# Autodesk Inventor assembly: Montagem1
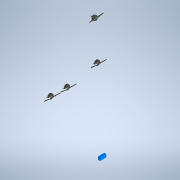
[picture p0: Inventor's stored thumbnail of the model, 180x180]
Saved by Autodesk Inventor 2022.6 (Build 266554000, 554)
## iProperties
Created: 2024-10-06
Part Number: Montagem1
Document SubType Name: Assembly
Designer: Olá
Author: Olá
## Documents named in this file (6)
- C:\Users\Olá\programacao\nasa\drone\Montagem1.iam
- C:\Users\Olá\programacao\nasa\drone\t-motor-u15-kv100-1.snapshot.2\U15 II KV 100\esc-motor-driver-t-motor-flame-80a-hv-6-12s-v2-1.snapshot.2\T-Motor Flame 80A HV 6-12S v2.ipt
- C:\Users\Olá\programacao\nasa\drone\t-motor-u15-kv100-1.snapshot.2\U15 II KV 100\t-motor-u15-kv100-1.snapshot.2\U15 II Kv 100.ipt
- C:\Users\Olá\programacao\nasa\drone\t-motor-u15-kv100-1.snapshot.2\U15 II KV 100\Hub.ipt
- C:\Users\Olá\programacao\nasa\drone\drone-propeller-10.snapshot.3\Drone propeller2.ipt
- C:\Users\Olá\programacao\nasa\drone\battery.ipt
## Components (17 placed, 5 different names)
1. T-Motor Flame 80A HV 6-12S v2:1
2. T-Motor Flame 80A HV 6-12S v2:2
3. T-Motor Flame 80A HV 6-12S v2:3
4. T-Motor Flame 80A HV 6-12S v2:4
5. U15 II Kv 100:2 — Coincidente:1, Coincidente:5, Coincidente:6, Coincidente:7, Coincidente:8
6. Hub:1 — Coincidente:5, Coincidente:6, Coincidente:8
7. Drone propeller2:1 — Coincidente:1, Coincidente:7
8. U15 II Kv 100:3
9. Hub:2
10. Drone propeller2:2
11. U15 II Kv 100:4
12. Hub:3
13. Drone propeller2:3
14. U15 II Kv 100:5
15. Hub:4
16. Drone propeller2:4
17. battery:1
## Relationships (20: Mate 20)
- Coincidente:1 [Mate]: U15 II Kv 100:2 ↔ Drone propeller2:1
- Coincidente:5 [Mate]: U15 II Kv 100:2 ↔ Hub:1
- Coincidente:6 [Mate]: U15 II Kv 100:2 ↔ Hub:1
- Coincidente:7 [Mate]: U15 II Kv 100:2 ↔ Drone propeller2:1
- Coincidente:8 [Mate]: U15 II Kv 100:2 ↔ Hub:1
- [Mate]: U15 II Kv 100:3 ↔ Drone propeller2:2
- [Mate]: U15 II Kv 100:3 ↔ Hub:2
- [Mate]: U15 II Kv 100:3 ↔ Hub:2
- [Mate]: U15 II Kv 100:3 ↔ Drone propeller2:2
- [Mate]: U15 II Kv 100:3 ↔ Hub:2
- [Mate]: U15 II Kv 100:4 ↔ Drone propeller2:3
- [Mate]: U15 II Kv 100:4 ↔ Hub:3
- [Mate]: U15 II Kv 100:4 ↔ Hub:3
- [Mate]: U15 II Kv 100:4 ↔ Drone propeller2:3
- [Mate]: U15 II Kv 100:4 ↔ Hub:3
- [Mate]: U15 II Kv 100:5 ↔ Drone propeller2:4
- [Mate]: U15 II Kv 100:5 ↔ Hub:4
- [Mate]: U15 II Kv 100:5 ↔ Hub:4
- [Mate]: U15 II Kv 100:5 ↔ Drone propeller2:4
- [Mate]: U15 II Kv 100:5 ↔ Hub:4
## Named parameters: d15_d0 = 0 mm, d16_d6 = 0 mm, d17_d7 = 0 mm, d18_d12 = 0 mm, d19_d13 = 16.3 mm, d20_d14 = 16.3 mm, d21_d9 = 0 mm, d22_d10 = 0.5 mm, d23_d11 = 0 mm, d24_d0 = 0 mm, d25_d6 = 0 mm, d26_d7 = 0 mm, d27_d12 = 0 mm, d28_d13 = 16.3 mm, d29_d14 = 16.3 mm, d30_d9 = 0 mm, d31_d10 = 0.5 mm, d32_d11 = 0 mm, d33_d0 = 0 mm, d34_d6 = 0 mm, d35_d7 = 0 mm, d36_d12 = 0 mm, d37_d13 = 16.3 mm, d38_d14 = 16.3 mm, d39_d9 = 0 mm, d40_d10 = 0.5 mm, d41_d11 = 0 mm
